# Autodesk Inventor assembly: ensambleSinFlanche
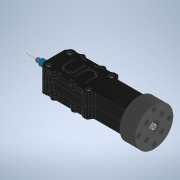
[picture p0: Inventor's stored thumbnail of the model, 180x180]
Saved by Autodesk Inventor 2021.5 (Build 255421000, 421)
## iProperties
Created: 2024-11-29
Part Number: ensambleSinFlanche
Document SubType Name: Assembly
Designer: Joho_
Mass: 143.945 g
Surface Area: 533.485 cm^2
Volume: 133.107 cm^3
Density: 1.08142 g/cm^3
Author: Joho_
## Documents named in this file (9)
- C:\Users\Joho_\Desktop\semestreN\robotica\laboratorios\lab01\CADs\ensambleSinFlanche.iam
- C:\Users\Joho_\Desktop\semestreN\robotica\laboratorios\lab01\CADs\baseSoporte.ipt
- C:\Users\Joho_\Desktop\semestreN\robotica\laboratorios\lab01\CADs\acople.ipt
- C:\Users\Joho_\Desktop\semestreN\robotica\laboratorios\lab01\CADs\marcador.ipt
- C:\Users\Joho_\Desktop\semestreN\robotica\laboratorios\lab01\CADs\tonrilloM3x20mm.ipt
- C:\Users\Joho_\Desktop\semestreN\robotica\laboratorios\lab01\CADs\tuercaM3.ipt
- C:\Users\Joho_\Desktop\semestreN\robotica\laboratorios\lab01\CADs\resorte5.ipt
- C:\Users\Joho_\Desktop\semestreN\robotica\laboratorios\lab01\CADs\tuercaM4.ipt
- C:\Users\Joho_\Desktop\semestreN\robotica\laboratorios\lab01\CADs\TornilloM4X20mm.ipt
## Components (23 placed, 8 different names)
1. baseSoporte:1 — Nivelación:1, Nivelación:2, Nivelación:3, Coincidencia:13, Coincidencia:14, Coincidencia:15, Coincidencia:16, Coincidencia:17, Coincidencia:20, Coincidencia:21, Coincidencia:24, Insertar:5
2. acople:1 — Coincidencia:1, Nivelación:4, Nivelación:5, Coincidencia:2, Nivelación:6, Insertar:1, Insertar:2, Insertar:3, Insertar:4, Coincidencia:11, Coincidencia:12, Coincidencia:19, Coincidencia:20
3. acople:2 — Coincidencia:1, Nivelación:4, Nivelación:5, Coincidencia:8, Coincidencia:9, Coincidencia:10, Coincidencia:18
4. marcador:1 — Coincidencia:2, Nivelación:6
5. tonrilloM3x20mm:1 — Insertar:1, Coincidencia:5
6. tonrilloM3x20mm:2 — Insertar:2, Coincidencia:6, Nivelación:16
7. tonrilloM3x20mm:3 — Insertar:3, Coincidencia:7
8. tonrilloM3x20mm:4 — Insertar:4, Coincidencia:3
9. tuercaM3:1 — Nivelación:7, Coincidencia:3
10. tuercaM3:2 — Nivelación:7, Nivelación:8, Coincidencia:5
11. tuercaM3:3 — Nivelación:8, Nivelación:9, Coincidencia:7
12. tuercaM3:4 — Nivelación:9, Coincidencia:6, Nivelación:16
13. tuercaM3:5 — Nivelación:11, Nivelación:12, Coincidencia:11
14. tuercaM3:6 — Nivelación:12, Coincidencia:12
15. tuercaM3:7 — Nivelación:10, Coincidencia:8, Coincidencia:9
16. tuercaM3:8 — Nivelación:10, Nivelación:11, Coincidencia:10
17. tonrilloM3x20mm:5 — Nivelación:13, Coincidencia:13, Coincidencia:19
18. tonrilloM3x20mm:6 — Nivelación:13, Nivelación:14, Coincidencia:16, Coincidencia:17, Coincidencia:18
19. tonrilloM3x20mm:7 — Nivelación:14, Nivelación:15, Coincidencia:15
20. tonrilloM3x20mm:8 — Nivelación:15, Coincidencia:14
21. resorte5:1 — Coincidencia:21, Coincidencia:22, Coincidencia:23, Coincidencia:24
22. tuercaM4:1 — Coincidencia:22, Coincidencia:23
23. TornilloM4X20mm:1 — Insertar:5
## Relationships (44: Mate 23, Flush 16, Insert 5)
- Nivelación:1 [Flush]: baseSoporte:1
- Nivelación:2 [Flush]: baseSoporte:1
- Nivelación:3 [Flush]: baseSoporte:1
- Coincidencia:1 [Mate]: acople:1 ↔ acople:2
- Nivelación:4 [Flush]: acople:1 ↔ acople:2
- Nivelación:5 [Flush]: acople:1 ↔ acople:2
- Coincidencia:2 [Mate]: acople:1 ↔ marcador:1
- Nivelación:6 [Flush]: acople:1 ↔ marcador:1
- Insertar:1 (1.5 mm): acople:1 ↔ tonrilloM3x20mm:1
- Insertar:2 (1.5 mm): acople:1 ↔ tonrilloM3x20mm:2
- Insertar:3 (1.5 mm): acople:1 ↔ tonrilloM3x20mm:3
- Insertar:4 (1.5 mm): acople:1 ↔ tonrilloM3x20mm:4
- Nivelación:7 [Flush]: tuercaM3:1 ↔ tuercaM3:2
- Nivelación:8 [Flush]: tuercaM3:2 ↔ tuercaM3:3
- Nivelación:9 [Flush]: tuercaM3:3 ↔ tuercaM3:4
- Coincidencia:3 [Mate]: tonrilloM3x20mm:4 ↔ tuercaM3:1
- Coincidencia:5 [Mate]: tonrilloM3x20mm:1 ↔ tuercaM3:2
- Coincidencia:6 [Mate]: tonrilloM3x20mm:2 ↔ tuercaM3:4
- Coincidencia:7 [Mate]: tonrilloM3x20mm:3 ↔ tuercaM3:3
- Nivelación:10 [Flush]: tuercaM3:7 ↔ tuercaM3:8
- Nivelación:11 [Flush]: tuercaM3:5 ↔ tuercaM3:8
- Nivelación:12 [Flush]: tuercaM3:5 ↔ tuercaM3:6
- Coincidencia:8 [Mate]: acople:2 ↔ tuercaM3:7
- Coincidencia:9 [Mate]: acople:2 ↔ tuercaM3:7
- Coincidencia:10 [Mate]: acople:2 ↔ tuercaM3:8
- Coincidencia:11 [Mate]: acople:1 ↔ tuercaM3:5
- Coincidencia:12 [Mate]: acople:1 ↔ tuercaM3:6
- Nivelación:13 [Flush]: tonrilloM3x20mm:5 ↔ tonrilloM3x20mm:6
- Nivelación:14 [Flush]: tonrilloM3x20mm:6 ↔ tonrilloM3x20mm:7
- Nivelación:15 [Flush]: tonrilloM3x20mm:7 ↔ tonrilloM3x20mm:8
- Coincidencia:13 [Mate]: baseSoporte:1 ↔ tonrilloM3x20mm:5
- Coincidencia:14 [Mate]: baseSoporte:1 ↔ tonrilloM3x20mm:8
- Coincidencia:15 [Mate]: baseSoporte:1 ↔ tonrilloM3x20mm:7
- Coincidencia:16 [Mate]: baseSoporte:1 ↔ tonrilloM3x20mm:6
- Coincidencia:17 [Mate]: baseSoporte:1 ↔ tonrilloM3x20mm:6
- Coincidencia:18 [Mate]: acople:2 ↔ tonrilloM3x20mm:6
- Nivelación:16 [Flush] (3.5 mm): tonrilloM3x20mm:2 ↔ tuercaM3:4
- Coincidencia:19 [Mate]: acople:1 ↔ tonrilloM3x20mm:5
- Coincidencia:20 [Mate]: baseSoporte:1 ↔ acople:1
- Coincidencia:21 [Mate]: baseSoporte:1 ↔ resorte5:1
- Coincidencia:22 [Mate]: resorte5:1 ↔ tuercaM4:1
- Coincidencia:23 [Mate]: resorte5:1 ↔ tuercaM4:1
- Coincidencia:24 [Mate]: baseSoporte:1 ↔ resorte5:1
- Insertar:5 (1 mm): baseSoporte:1 ↔ TornilloM4X20mm:1
